# Autodesk Inventor assembly: Flex_Giubo_Assembly
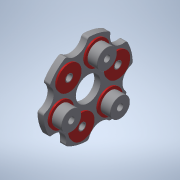
[picture p0: Inventor's stored thumbnail of the model, 180x180]
Saved by Autodesk Inventor 2021 (Build 250183000, 183)
## iProperties
Created: 2020-10-13
Part Number: Flex_Giubo_Assembly
Document SubType Name: Assembly
Designer: PhotonUser
Quantity: 1
Author: PhotonUser
## Documents named in this file (5)
- D:\PhotonUser\Downloads\Assembly Files-20201111T001656Z-001\Assembly Files\Flex_Giubo_Assembly.iam
- D:\PhotonUser\Downloads\Assembly Files-20201111T001656Z-001\Assembly Files\Poly_Bushing.ipt
- D:\PhotonUser\Downloads\Assembly Files-20201111T001656Z-001\Assembly Files\Flex_Giubo_V1.ipt
- D:\PhotonUser\Downloads\Assembly Files-20201111T001656Z-001\Assembly Files\Flex_Bushing.ipt
- D:\PhotonUser\Downloads\Assembly Files-20201111T001656Z-001\Assembly Files\Flex_Bushing_NONSPACER.ipt
## Components (19 placed, 4 different names)
1. Poly_Bushing:1 — Insert:4
2. Poly_Bushing:3 — Insert:6
3. Poly_Bushing:4 — Insert:3
4. Poly_Bushing:5 — Insert:2
5. Poly_Bushing:7 — Insert:7
6. Flex_Giubo_V1:1 — Insert:2, Insert:3, Insert:4, Insert:6, Insert:7, Insert:8, Insert:9, Insert:10, Insert:11, Insert:12, Insert:13, Insert:14
7. Poly_Bushing:8 — Insert:9, Insert:17
8. Poly_Bushing:9 — Insert:13, Insert:20
9. Poly_Bushing:10 — Insert:14
10. Poly_Bushing:11 — Insert:12, Insert:16
11. Poly_Bushing:12 — Insert:11, Insert:19
12. Poly_Bushing:13 — Insert:10, Insert:15
13. Poly_Bushing:14 — Insert:8, Insert:18
14. Flex_Bushing:1 — Insert:16
15. Flex_Bushing:2 — Insert:17
16. Flex_Bushing:3 — Insert:15
17. Flex_Bushing_NONSPACER:1 — Insert:19
18. Flex_Bushing_NONSPACER:2 — Insert:20
19. Flex_Bushing_NONSPACER:3 — Insert:18
## Relationships (18: Insert 18)
- Insert:2: Poly_Bushing:5 ↔ Flex_Giubo_V1:1
- Insert:3: Poly_Bushing:4 ↔ Flex_Giubo_V1:1
- Insert:4: Poly_Bushing:1 ↔ Flex_Giubo_V1:1
- Insert:6: Poly_Bushing:3 ↔ Flex_Giubo_V1:1
- Insert:7: Poly_Bushing:7 ↔ Flex_Giubo_V1:1
- Insert:8: Flex_Giubo_V1:1 ↔ Poly_Bushing:14
- Insert:9: Flex_Giubo_V1:1 ↔ Poly_Bushing:8
- Insert:10: Flex_Giubo_V1:1 ↔ Poly_Bushing:13
- Insert:11: Flex_Giubo_V1:1 ↔ Poly_Bushing:12
- Insert:12: Flex_Giubo_V1:1 ↔ Poly_Bushing:11
- Insert:13: Flex_Giubo_V1:1 ↔ Poly_Bushing:9
- Insert:14: Flex_Giubo_V1:1 ↔ Poly_Bushing:10
- Insert:15: Poly_Bushing:13 ↔ Flex_Bushing:3
- Insert:16: Poly_Bushing:11 ↔ Flex_Bushing:1
- Insert:17: Poly_Bushing:8 ↔ Flex_Bushing:2
- Insert:18: Poly_Bushing:14 ↔ Flex_Bushing_NONSPACER:3
- Insert:19: Poly_Bushing:12 ↔ Flex_Bushing_NONSPACER:1
- Insert:20: Poly_Bushing:9 ↔ Flex_Bushing_NONSPACER:2
